# Autodesk Inventor assembly: SteelM-StarS_mirrored
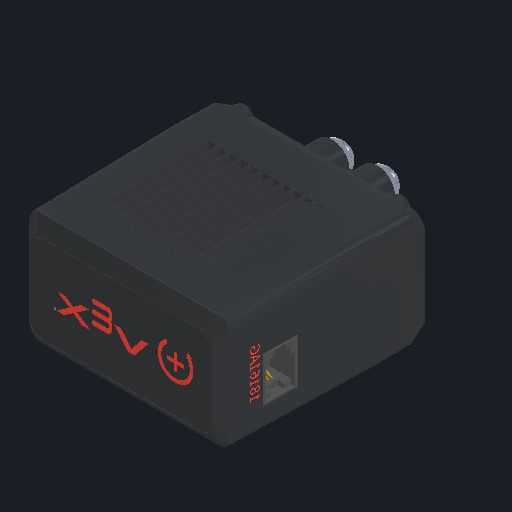
[picture p0: Inventor's stored thumbnail of the model, 512x512]
Saved by Autodesk Inventor 2025 (Build 290162000, 162)
## iProperties
Created: 2022-08-18
Part Number: SteelM-StarS_mirrored
Document SubType Name: Assembly
Designer: Averey Ku
Author: ylu12
## Documents named in this file (4)
- D:\vex_robotics_high_stakes\hardware\cad\EARLY_SEASON\chassis\mirrored_parts\SteelM-StarS_mirrored.iam
- D:\vex_robotics_high_stakes\hardware\cad\EARLY_SEASON\chassis\mirrored_parts\V5 Motor_mirrored.ipt
- D:\vex_robotics_high_stakes\hardware\cad\VEX-CAD-Inventor\Structure\Hardware\Screw Steel - Star\SScrew Star Smooth .500.ipt
- D:\vex_robotics_high_stakes\hardware\cad\VEX-CAD-Inventor\Structure\Hardware\Screw Steel - Star.ipt
## Components (3 placed, 2 different names)
1. V5 Motor_mirrored:1
2. SScrew Star Smooth .500:1
3. SScrew Star Smooth .500:2
## Named parameters: Thickness = 1.1938 mm
